# Autodesk Inventor assembly: czujnik zalania v3
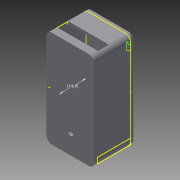
[picture p0: Inventor's stored thumbnail of the model, 180x180]
Saved by Autodesk Inventor 2014 (Build 180170000, 170)
## iProperties
Created: 2018-03-27
Part Number: czujnik zalania v3
Document SubType Name: Assembly
Designer: HP820
Author: HP820
## Documents named in this file (3)
- C:\Users\HP820\Dysk Google\Projekt SYSTEM POWIADOMIEN DLA OSOB GLUCHONIEMYCH I NIEDOSLYSZACYCH BY JACEK MARTYNIAK I ŁUKASZ NOWARKIEWICZ\Projekty 3D obudowy\czujnik zalania\czujnik zalania v3.iam
- C:\Users\HP820\Dysk Google\Projekt SYSTEM POWIADOMIEN DLA OSOB GLUCHONIEMYCH I NIEDOSLYSZACYCH BY JACEK MARTYNIAK I ŁUKASZ NOWARKIEWICZ\Projekty 3D obudowy\czujnik zalania\bottom v3.ipt
- C:\Users\HP820\Dysk Google\Projekt SYSTEM POWIADOMIEN DLA OSOB GLUCHONIEMYCH I NIEDOSLYSZACYCH BY JACEK MARTYNIAK I ŁUKASZ NOWARKIEWICZ\Projekty 3D obudowy\czujnik zalania\top v3.ipt
## Components (2 placed, 2 different names)
1. bottom v3:1 — Flush:1
2. top v3:1 — Flush:1
## Relationships (1: Flush 1)
- Flush:1: bottom v3:1 ↔ top v3:1
